# Autodesk Inventor assembly: CrossRail
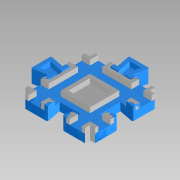
[picture p0: Inventor's stored thumbnail of the model, 180x180]
Saved by Autodesk Inventor 2021 (Build 250183000, 183)
## iProperties
Created: 2021-05-27
Part Number: CrossRail
Document SubType Name: Assembly
Designer: kumagai
Author: kumagai
## Documents named in this file (5)
- X:\Develop\CAD\PlaRails\DoubleSlip\CrossRail.iam
- X:\Develop\CAD\PlaRails\DoubleSlip\CrossRail\CrossRail-DSS.ipt
- X:\Develop\CAD\PlaRails\DoubleSlip\CrossRail.ipt
- X:\Develop\CAD\PlaRails\DoubleSlip\RailJointShortMale_filled.ipt
- X:\Develop\CAD\PlaRails\DoubleSlip\RailJointShortFemale_filled.ipt
## Components (5 placed, 3 different names)
1. CrossRail-DSS:1 — フラッシュ:1, フラッシュ:2, フラッシュ:3, フラッシュ:4, フラッシュ:5, メイト:1, フラッシュ:6, フラッシュ:7, フラッシュ:8, メイト:2, メイト:3, メイト:4
2. RailJointShortMale_filled:1 — フラッシュ:1, フラッシュ:6, メイト:3
3. RailJointShortMale_filled:2 — フラッシュ:2, フラッシュ:7, メイト:4
4. RailJointShortFemale_filled:1 — フラッシュ:4, フラッシュ:8, メイト:2
5. RailJointShortFemale_filled:2 — フラッシュ:3, フラッシュ:5, メイト:1
## Relationships (12: Flush 8, Mate 4)
- フラッシュ:1 [Flush]: CrossRail-DSS:1 ↔ RailJointShortMale_filled:1
- フラッシュ:2 [Flush]: CrossRail-DSS:1 ↔ RailJointShortMale_filled:2
- フラッシュ:3 [Flush]: CrossRail-DSS:1 ↔ RailJointShortFemale_filled:2
- フラッシュ:4 [Flush]: CrossRail-DSS:1 ↔ RailJointShortFemale_filled:1
- フラッシュ:5 [Flush]: CrossRail-DSS:1 ↔ RailJointShortFemale_filled:2
- メイト:1 [Mate]: CrossRail-DSS:1 ↔ RailJointShortFemale_filled:2
- フラッシュ:6 [Flush]: CrossRail-DSS:1 ↔ RailJointShortMale_filled:1
- フラッシュ:7 [Flush]: CrossRail-DSS:1 ↔ RailJointShortMale_filled:2
- フラッシュ:8 [Flush]: CrossRail-DSS:1 ↔ RailJointShortFemale_filled:1
- メイト:2 [Mate]: CrossRail-DSS:1 ↔ RailJointShortFemale_filled:1
- メイト:3 [Mate]: CrossRail-DSS:1 ↔ RailJointShortMale_filled:1
- メイト:4 [Mate]: CrossRail-DSS:1 ↔ RailJointShortMale_filled:2
